# Autodesk Inventor assembly: Reactor_SOLID_Nowrist
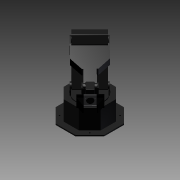
[picture p0: Inventor's stored thumbnail of the model, 180x180]
Saved by Autodesk Inventor 2012 (Build 160160000, 160)
## iProperties
Created: 2013-02-21
Part Number: Reactor_SOLID_Nowrist
Document SubType Name: Assembly
Designer: Andrew
Author: Andrew
## Documents named in this file (7)
- R:\PhantomX Reactor Arm\Reactor_SOLID\Reactor_SOLID_Nowrist.iam
- R:\PhantomX Reactor Arm\Reactor_SOLID\Base.ipt
- R:\PhantomX Reactor Arm\Reactor_SOLID\Shoulder.ipt
- R:\PhantomX Reactor Arm\Reactor_SOLID\Bicep.ipt
- R:\PhantomX Reactor Arm\Reactor_SOLID\ForeArm.ipt
- R:\PhantomX Reactor Arm\Reactor_SOLID\Wrist.ipt
- R:\PhantomX Reactor Arm\Reactor_SOLID\Imported Components\PX-Gripper\PX-Gripper.iam
## Components (6 placed, 6 different names)
1. Base:1 — Insert:1, Angle:1
2. Shoulder:1 — Insert:1, Insert:7
3. Bicep:1 — Insert:7, Insert:8
4. ForeArm:1 — Insert:8, Insert:9
5. Wrist:1 — Angle:1, Insert:9, Insert:10, Angle:2
6. PX-Gripper:1 [sub-assembly] — Insert:10, Angle:2
## Relationships (7: Insert 5, Angle 2)
- Insert:1: Base:1 ↔ Shoulder:1
- Angle:1 (0 deg): Base:1 ↔ Wrist:1
- Insert:7: Shoulder:1 ↔ Bicep:1
- Insert:8: Bicep:1 ↔ ForeArm:1
- Insert:9: ForeArm:1 ↔ Wrist:1
- Insert:10: Wrist:1 ↔ PX-Gripper:1
- Angle:2 (0 deg): Wrist:1 ↔ PX-Gripper:1
